# Autodesk Inventor assembly: Assembly1
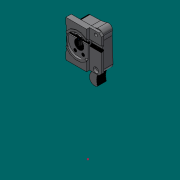
[picture p0: Inventor's stored thumbnail of the model, 180x180]
Saved by Autodesk Inventor 2018 (Build 220112000, 112)
## iProperties
Created: 2020-10-19
Part Number: Assembly1
Material: 一般
Document SubType Name: Assembly
Designer: gisen
Author: gisen
## Documents named in this file (3)
- C:\Users\gisen\Documents\CAD\inventor\git\upbox_extruder_unit\knob\Assembly1.iam
- C:\Users\gisen\Documents\CAD\inventor\git\upbox_extruder_unit\knob\Body_v2.ipt
- C:\Users\gisen\Documents\CAD\inventor\git\upbox_extruder_unit\knob\leaver_v2.ipt
## Components (2 placed, 2 different names)
1. Body_v2:1 — メイト:1, メイト:2
2. leaver_v2:1 — メイト:1, メイト:2
## Relationships (2: Mate 2)
- メイト:1 [Mate]: Body_v2:1 ↔ leaver_v2:1
- メイト:2 [Mate] (0.5 mm): Body_v2:1 ↔ leaver_v2:1
